# Autodesk Inventor assembly: Overall_Assembly
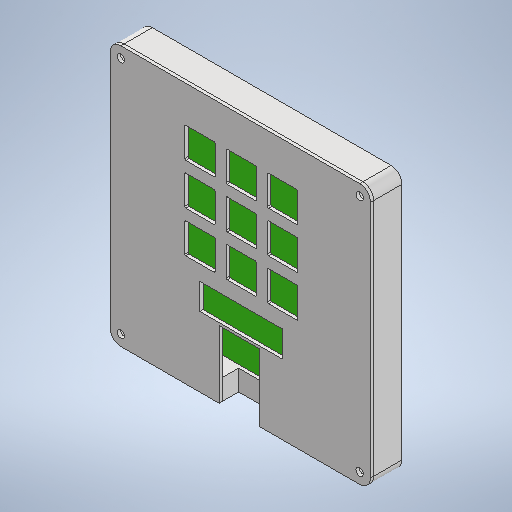
[picture p0: Inventor's stored thumbnail of the model, 512x512]
Saved by Autodesk Inventor 2025.1 (Build 291241000, 241)
## iProperties
Created: 2025-12-17
Part Number: Overall_Assembly
Document SubType Name: Assembly
Designer: omara
Author: omara
## Documents named in this file (4)
- C:\Users\omara\Desktop\Macropad_Project\Overall_Assembly.iam
- C:\Users\omara\Desktop\Macropad_Project\Bottom_Case_New.ipt
- C:\Users\omara\Desktop\Macropad_Project\PCB_Plate.ipt
- C:\Users\omara\Desktop\Macropad_Project\Top_Case_New.ipt
## Components (3 placed, 3 different names)
1. Bottom_Case_New:1 — Mate:1, Mate:2, Mate:3, Insert:1, Insert:2
2. PCB_Plate:1 — Mate:1, Mate:2, Mate:3
3. Top_Case_New:1 — Insert:1, Insert:2
## Relationships (5: Mate 3, Insert 2)
- Mate:1: Bottom_Case_New:1 ↔ PCB_Plate:1
- Mate:2: Bottom_Case_New:1 ↔ PCB_Plate:1
- Mate:3: Bottom_Case_New:1 ↔ PCB_Plate:1
- Insert:1: Bottom_Case_New:1 ↔ Top_Case_New:1
- Insert:2: Bottom_Case_New:1 ↔ Top_Case_New:1
